# Autodesk Inventor assembly: Remote Assembly
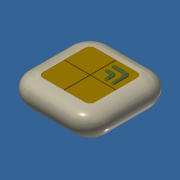
[picture p0: Inventor's stored thumbnail of the model, 180x180]
Saved by Autodesk Inventor 2016 (Build 200138000, 138)
## iProperties
Created: 2015-06-16
Part Number: Remote Assembly
Document SubType Name: Assembly
Designer: Samuel Clay
Author: Samuel Clay
## Documents named in this file (8)
- Z:\enclosure\inventor\Remote Assembly.iam
- Z:\enclosure\inventor\Remote Top.ipt
- Z:\enclosure\inventor\Remote Bottom.ipt
- Z:\enclosure\inventor\Remote Buttons.ipt
- Z:\enclosure\inventor\Eagle PCB rev 21.ipt
- Z:\enclosure\inventor\Case Bottom.ipt
- Z:\enclosure\inventor\Case Top.ipt
- Z:\enclosure\inventor\Case Buttons.ipt
## Components (7 placed, 7 different names)
1. Case Top:1 — Mate:3
2. Remote Top:1 — Flush:1, Mate:1, Mate:3
3. Case Buttons:1 — Mate:2
4. Remote Buttons:1 — Flush:1, Mate:1, Mate:2
5. Eagle PCB rev 21:1 — Rotational:1
6. Remote Bottom:1 — Rotational:1
7. Case Bottom:1
## Relationships (5: Mate 3, Flush 1, RevoluteJoint 1)
- Flush:1: Remote Top:1 ↔ Remote Buttons:1
- Mate:1: Remote Top:1 ↔ Remote Buttons:1
- Mate:2: Case Buttons:1 ↔ Remote Buttons:1
- Mate:3: Case Top:1 ↔ Remote Top:1
- Rotational:1 [RevoluteJoint]: Eagle PCB rev 21:1 ↔ Remote Bottom:1
